# Autodesk Inventor assembly: エンコーダ取り付け
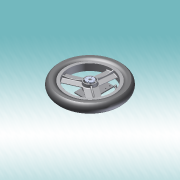
[picture p0: Inventor's stored thumbnail of the model, 180x180]
Saved by Autodesk Inventor 2015 (Build 190159000, 159)
## iProperties
Created: 2016-02-18
Part Number: エンコーダ取り付け
Document SubType Name: Assembly
Designer: buzztaka
Author: buzztaka
## Documents named in this file (8)
- C:\Users\buzztaka\Documents\tukuba\i-cart-middle_3d-model\計測輪アセンブル\エンコーダ取り付け.iam
- C:\Users\buzztaka\Documents\tukuba\i-cart-middle_3d-model\計測輪アセンブル\スプリングフランジ.ipt
- C:\Users\buzztaka\Documents\tukuba\i-cart-middle_3d-model\計測輪アセンブル\meh-30-pエンコーダ.ipt
- C:\Users\buzztaka\Documents\tukuba\i-cart-middle_3d-model\計測輪アセンブル\エンコーダ取り付け板.ipt
- C:\Users\buzztaka\Documents\tukuba\i-cart-middle_3d-model\計測輪アセンブル\wheel_12inch.ipt
- C:\Users\buzztaka\Documents\tukuba\i-cart-middle_3d-model\計測輪アセンブル\wheel-hub.ipt
- C:\Users\buzztaka\Documents\tukuba\i-cart-middle_3d-model\計測輪アセンブル\whelelcapholl.ipt
- C:\Users\buzztaka\Documents\tukuba\i-cart-middle_3d-model\計測輪アセンブル\正しい.ipt
## Components (7 placed, 7 different names)
1. meh-30-pエンコーダ:1 — 挿入:1, 挿入:2, 挿入:12
2. スプリングフランジ:1 — 挿入:1, 挿入:2, 挿入:4
3. エンコーダ取り付け板:1 — 挿入:4
4. wheel_12inch:1 — 挿入:7, 挿入:8, 挿入:9, 挿入:10
5. wheel-hub:1 — 挿入:7, 挿入:8
6. whelelcapholl:1 — 挿入:9, 挿入:10, 挿入:11
7. 正しい:1 — 挿入:11, 挿入:12
## Relationships (9: Insert 9)
- 挿入:1 [Insert]: meh-30-pエンコーダ:1 ↔ スプリングフランジ:1
- 挿入:2 [Insert]: meh-30-pエンコーダ:1 ↔ スプリングフランジ:1
- 挿入:4 [Insert]: スプリングフランジ:1 ↔ エンコーダ取り付け板:1
- 挿入:7 [Insert]: wheel_12inch:1 ↔ wheel-hub:1
- 挿入:8 [Insert]: wheel_12inch:1 ↔ wheel-hub:1
- 挿入:9 [Insert]: wheel_12inch:1 ↔ whelelcapholl:1
- 挿入:10 [Insert]: wheel_12inch:1 ↔ whelelcapholl:1
- 挿入:11 [Insert]: whelelcapholl:1 ↔ 正しい:1
- 挿入:12 [Insert] (-10 mm): meh-30-pエンコーダ:1 ↔ 正しい:1
